# Autodesk Inventor assembly: CNC-FullAssembly
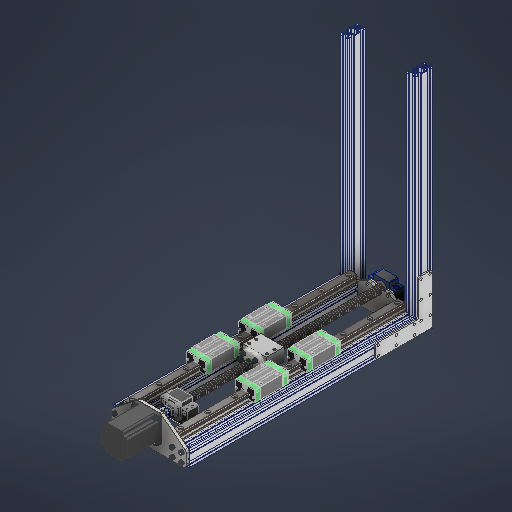
[picture p0: Inventor's stored thumbnail of the model, 512x512]
Saved by Autodesk Inventor 2026.2 (Build 302298000, 298)
## iProperties
Created: 2026-06-14
Part Number: CNC-FullAssembly
Document SubType Name: Assembly
Designer: Kenji
Mass: 7911.16 g
Surface Area: 12466.7 cm^2
Volume: 1822.96 cm^3
Density: 4.33972 g/cm^3
Author: Kenji
## Documents named in this file (20)
- C:\Users\Kenji\Documents\GitHub\DiyCNC-\CNC-FullAssembly.iam
- C:\Users\Kenji\Documents\GitHub\DiyCNC-\COTS-Parts\40x40x500mm-Extrusion.ipt
- C:\Users\Kenji\Documents\GitHub\DiyCNC-\COTS-Parts\SFU1605-BallScrewNut.iam
- C:\Users\Kenji\Documents\GitHub\DiyCNC-\COTS-Parts\DSG16H-BallScrewFixtureBlock.ipt
- C:\Users\Kenji\Documents\GitHub\DiyCNC-\COTS-Parts\SFU1605-BallScrew500mm.ipt
- C:\Users\Kenji\Documents\GitHub\DiyCNC-\COTS-Parts\BK12-BallScrewStabilizer.iam
- C:\Users\Kenji\Documents\GitHub\DiyCNC-\COTS-Parts\HGR20R-LinearRail500mm.ipt
- C:\Users\Kenji\Documents\GitHub\DiyCNC-\COTS-Parts\HGH20-LinearRailCarriage.iam
- C:\Users\Kenji\Documents\GitHub\DiyCNC-\COTS-Parts\91274A131_M5x20mm.ipt
- C:\Users\Kenji\Documents\GitHub\DiyCNC-\COTS-Parts\91290A231-M5x15mm.ipt
- C:\Users\Kenji\Documents\GitHub\DiyCNC-\COTS-Parts\Nema23-StepperMotor.ipt
- C:\Users\Kenji\Documents\GitHub\DiyCNC-\COTS-Parts\MH2025-6.35x10mmCoupler.iam
- C:\Users\Kenji\Documents\GitHub\DiyCNC-\COTS-Parts\BF12-BallScrewStabilizer2.ipt
- C:\Users\Kenji\Documents\GitHub\DiyCNC-\CNC-000-StructureGusset1.ipt
- C:\Users\Kenji\Documents\GitHub\DiyCNC-\COTS-Parts\20x40x500mm-Extrusion.ipt
- C:\Users\Kenji\Documents\GitHub\DiyCNC-\CNC-001-StructureGusset2.ipt
- C:\Users\Kenji\Documents\GitHub\DiyCNC-\CNC-002-ShimStructureGusset2.ipt
- C:\Users\Kenji\Documents\GitHub\DiyCNC-\COTS-Parts\90576A104-M5-NylockNut.ipt
- C:\Users\Kenji\Documents\GitHub\DiyCNC-\COTS-Parts\91292A195-M5x45mm.ipt
- C:\Users\Kenji\Documents\GitHub\DiyCNC-\CNC-003-StructureGusset3.ipt
## Components (70 placed, 19 different names)
1. 40x40x500mm-Extrusion:1 — Mate:1, Mate:2, Flush:1, Flush:2, Flush:3, Angle:1, Mate:6, Mate:12, Flush:5, Flush:6, Angle:3, Angle:4, Mate:46, Flush:20, Flush:21, Mate:48, Mate:49, Mate:50, Flush:35
2. 40x40x500mm-Extrusion:2 — Flush:2, Flush:3, Mate:7, Angle:2, Mate:11, Flush:9, Mate:39, Mate:40, Mate:41, Flush:22, Mate:47, Flush:23, Flush:38
3. SFU1605-BallScrewNut:1 [sub-assembly] — Mate:3, Mate:4, Mate:5, Mate:8, Mate:21, Mate:22, Mate:23, Mate:24, Mate:25, Mate:26, Mate:27
4. DSG16H-BallScrewFixtureBlock:1 — Mate:3, Mate:4, Mate:5, Angle:1, Mate:6, Mate:7, Flush:14, Mate:20
5. SFU1605-BallScrew500mm:1 — Mate:8, Mate:9, Mate:10, Mate:30, Mate:34, Mate:35, Mate:36
6. BK12-BallScrewStabilizer:1 [sub-assembly] — Mate:9, Mate:10, Angle:2
7. HGR20R-LinearRail500mm:1 — Mate:12, Flush:5, Flush:6, Flush:7, Flush:8, Mate:13, Mate:14, Mate:17, Mate:28, Mate:29, Mate:37
8. HGR20R-LinearRail500mm:2 — Mate:11, Flush:7, Flush:8, Flush:9, Mate:15, Mate:16, Mate:19
9. HGH20-LinearRailCarriage:1 [sub-assembly] — Mate:13, Mate:14, Flush:10, Flush:11, Mate:18, Flush:14
10. HGH20-LinearRailCarriage:2 [sub-assembly] — Mate:19, Flush:12, Flush:13
11. HGH20-LinearRailCarriage:3 [sub-assembly] — Mate:15, Mate:16, Flush:10, Flush:12, Mate:20
12. HGH20-LinearRailCarriage:4 [sub-assembly] — Mate:17, Flush:11, Mate:18, Flush:13
13. 91274A131_M5x20mm:1 — Mate:21, Mate:22, Flush:17, Flush:18
14. 91274A131_M5x20mm:2 — Mate:26, Flush:15, Flush:16
15. 91274A131_M5x20mm:3 — Mate:27, Flush:15
16. 91274A131_M5x20mm:4 — Mate:25, Flush:16, Flush:17
17. 91274A131_M5x20mm:5 — Mate:23, Flush:18, Flush:19
18. 91274A131_M5x20mm:6 — Mate:24, Flush:19
19. Nema23-StepperMotor:1 — Mate:32, Angle:3, Mate:33, Mate:59, Mate:60, Mate:61, Mate:62, Mate:63
20. MH2025-6.35x10mmCoupler:1 [sub-assembly] — Mate:30, Mate:32, Mate:33, Mate:34
21. BF12-BallScrewStabilizer2:1 — Mate:35, Mate:36, Angle:4, Mate:37, Mate:56, Mate:57, Mate:58
22. CNC-000-StructureGusset1:1 — Mate:39, Mate:40, Mate:41, Mate:42, Mate:43, Mate:44, Mate:45, Mate:65
23. 20x40x500mm-Extrusion:1 — Mate:46, Flush:20, Flush:21, Mate:71, Mate:72, Mate:73, Mate:74, Mate:75, Flush:36
24. 20x40x500mm-Extrusion:2 — Flush:22, Mate:47, Flush:23, Mate:69, Mate:70, Mate:76, Flush:37
25. CNC-001-StructureGusset2:1 — Mate:48, Mate:49, Mate:50, Mate:51, Mate:52, Mate:53, Mate:54, Mate:55
26. 91290A231-M5x15mm:27 — Mate:51, Mate:52, Flush:25, Flush:26
27. 91290A231-M5x15mm:28 — Mate:54, Flush:24, Flush:25
28. 91290A231-M5x15mm:29 — Mate:55, Flush:24
29. 91290A231-M5x15mm:30 — Mate:53, Flush:26
30. CNC-002-ShimStructureGusset2:1 — Mate:56, Mate:57, Mate:58
31. 91274A131_M5x20mm:7 — Mate:60, Flush:29, Mate:67
32. 91274A131_M5x20mm:8 — Mate:62, Mate:63, Flush:27, Mate:68
33. 91274A131_M5x20mm:9 — Mate:59, Flush:28, Flush:29, Mate:64
34. 91274A131_M5x20mm:10 — Mate:61, Flush:27, Flush:28, Mate:66
35. 90576A104-M5-NylockNut:1 — Mate:64, Mate:65, Flush:32
36. 90576A104-M5-NylockNut:2 — Mate:66, Flush:30
37. 90576A104-M5-NylockNut:3 — Mate:68, Flush:30, Flush:31
38. 90576A104-M5-NylockNut:4 — Mate:67, Flush:31, Flush:32
39. 91292A195-M5x45mm:1 — Mate:69, Flush:33, Flush:34
40. 91292A195-M5x45mm:2 — Mate:70, Flush:34
41. 91292A195-M5x45mm:3 — Mate:72, Mate:73
42. 91292A195-M5x45mm:4 — Mate:71, Mate:74, Flush:33
43. CNC-003-StructureGusset3:1 — Mate:75, Flush:35, Flush:36
44. CNC-003-StructureGusset3:2 — Mate:76, Flush:37, Flush:38
45. 91290A231-M5x15mm:1 — Mate:28, Mate:29
46. 91290A231-M5x15mm:2
47. 91290A231-M5x15mm:3
48. 91290A231-M5x15mm:4
49. 91290A231-M5x15mm:5
50. 91290A231-M5x15mm:6
51. 91290A231-M5x15mm:7
52. 91290A231-M5x15mm:8
53. 91290A231-M5x15mm:9
54. 91290A231-M5x15mm:10
55. 91290A231-M5x15mm:11
56. 91290A231-M5x15mm:12
57. 91290A231-M5x15mm:13
58. 91290A231-M5x15mm:14
59. 91290A231-M5x15mm:15
60. 91290A231-M5x15mm:16
61. 91290A231-M5x15mm:17
62. 91290A231-M5x15mm:18
63. 91290A231-M5x15mm:20 — Mate:44, Mate:45
64. 91290A231-M5x15mm:21
65. 91290A231-M5x15mm:22
66. 91290A231-M5x15mm:23
67. 91290A231-M5x15mm:19 — Mate:42, Mate:43
68. 91290A231-M5x15mm:24
69. 91290A231-M5x15mm:25
70. 91290A231-M5x15mm:26
## Component patterns: (18 elements, first: 91290A231-M5x15mm:1), (4 elements, first: 91290A231-M5x15mm:20), (4 elements, first: 91290A231-M5x15mm:19)
## Relationships (115: Mate 74, Flush 37, Angle 4)
- Mate:1 (-20 mm): 40x40x500mm-Extrusion:1
- Mate:2 (-20 mm): 40x40x500mm-Extrusion:1
- Flush:1 (-250 mm): 40x40x500mm-Extrusion:1
- Flush:2: 40x40x500mm-Extrusion:1 ↔ 40x40x500mm-Extrusion:2
- Flush:3: 40x40x500mm-Extrusion:1 ↔ 40x40x500mm-Extrusion:2
- Mate:3: SFU1605-BallScrewNut:1 ↔ DSG16H-BallScrewFixtureBlock:1
- Mate:4: SFU1605-BallScrewNut:1 ↔ DSG16H-BallScrewFixtureBlock:1
- Mate:5: SFU1605-BallScrewNut:1 ↔ DSG16H-BallScrewFixtureBlock:1
- Angle:1 (0 deg): 40x40x500mm-Extrusion:1 ↔ DSG16H-BallScrewFixtureBlock:1
- Mate:6 (18 mm): 40x40x500mm-Extrusion:1 ↔ DSG16H-BallScrewFixtureBlock:1
- Mate:7 (18 mm): 40x40x500mm-Extrusion:2 ↔ DSG16H-BallScrewFixtureBlock:1
- Mate:8: SFU1605-BallScrewNut:1 ↔ SFU1605-BallScrew500mm:1
- Mate:9: SFU1605-BallScrew500mm:1 ↔ BK12-BallScrewStabilizer:1
- Mate:10: SFU1605-BallScrew500mm:1 ↔ BK12-BallScrewStabilizer:1
- Angle:2 (0 deg): 40x40x500mm-Extrusion:2 ↔ BK12-BallScrewStabilizer:1
- Mate:11: 40x40x500mm-Extrusion:2 ↔ HGR20R-LinearRail500mm:2
- Mate:12: 40x40x500mm-Extrusion:1 ↔ HGR20R-LinearRail500mm:1
- Flush:5: 40x40x500mm-Extrusion:1 ↔ HGR20R-LinearRail500mm:1
- Flush:6: 40x40x500mm-Extrusion:1 ↔ HGR20R-LinearRail500mm:1
- Flush:7: HGR20R-LinearRail500mm:1 ↔ HGR20R-LinearRail500mm:2
- Flush:8: HGR20R-LinearRail500mm:1 ↔ HGR20R-LinearRail500mm:2
- Flush:9: 40x40x500mm-Extrusion:2 ↔ HGR20R-LinearRail500mm:2
- Mate:13: HGR20R-LinearRail500mm:1 ↔ HGH20-LinearRailCarriage:1
- Mate:14: HGR20R-LinearRail500mm:1 ↔ HGH20-LinearRailCarriage:1
- Mate:15: HGR20R-LinearRail500mm:2 ↔ HGH20-LinearRailCarriage:3
- Mate:16: HGR20R-LinearRail500mm:2 ↔ HGH20-LinearRailCarriage:3
- Flush:10: HGH20-LinearRailCarriage:1 ↔ HGH20-LinearRailCarriage:3
- Mate:17: HGR20R-LinearRail500mm:1 ↔ HGH20-LinearRailCarriage:4
- Flush:11: HGH20-LinearRailCarriage:1 ↔ HGH20-LinearRailCarriage:4
- Mate:18 (40 mm): HGH20-LinearRailCarriage:1 ↔ HGH20-LinearRailCarriage:4
- Mate:19: HGR20R-LinearRail500mm:2 ↔ HGH20-LinearRailCarriage:2
- Flush:12: HGH20-LinearRailCarriage:2 ↔ HGH20-LinearRailCarriage:3
- Flush:13: HGH20-LinearRailCarriage:2 ↔ HGH20-LinearRailCarriage:4
- Flush:14: DSG16H-BallScrewFixtureBlock:1 ↔ HGH20-LinearRailCarriage:1
- Mate:20: DSG16H-BallScrewFixtureBlock:1 ↔ HGH20-LinearRailCarriage:3
- Mate:21: SFU1605-BallScrewNut:1 ↔ 91274A131_M5x20mm:1
- Mate:22: SFU1605-BallScrewNut:1 ↔ 91274A131_M5x20mm:1
- Mate:23: SFU1605-BallScrewNut:1 ↔ 91274A131_M5x20mm:5
- Mate:24: SFU1605-BallScrewNut:1 ↔ 91274A131_M5x20mm:6
- Mate:25: SFU1605-BallScrewNut:1 ↔ 91274A131_M5x20mm:4
- Mate:26: SFU1605-BallScrewNut:1 ↔ 91274A131_M5x20mm:2
- Mate:27: SFU1605-BallScrewNut:1 ↔ 91274A131_M5x20mm:3
- Flush:15: 91274A131_M5x20mm:2 ↔ 91274A131_M5x20mm:3
- Flush:16: 91274A131_M5x20mm:2 ↔ 91274A131_M5x20mm:4
- Flush:17: 91274A131_M5x20mm:1 ↔ 91274A131_M5x20mm:4
- Flush:18: 91274A131_M5x20mm:1 ↔ 91274A131_M5x20mm:5
- Flush:19: 91274A131_M5x20mm:5 ↔ 91274A131_M5x20mm:6
- Mate:28: HGR20R-LinearRail500mm:1 ↔ 91290A231-M5x15mm:1
- Mate:29: HGR20R-LinearRail500mm:1 ↔ 91290A231-M5x15mm:1
- Mate:30: SFU1605-BallScrew500mm:1 ↔ MH2025-6.35x10mmCoupler:1
- Mate:32: Nema23-StepperMotor:1 ↔ MH2025-6.35x10mmCoupler:1
- Angle:3 (0 deg): 40x40x500mm-Extrusion:1 ↔ Nema23-StepperMotor:1
- Mate:33 (2 mm): Nema23-StepperMotor:1 ↔ MH2025-6.35x10mmCoupler:1
- Mate:34 (2 mm): SFU1605-BallScrew500mm:1 ↔ MH2025-6.35x10mmCoupler:1
- Mate:35: SFU1605-BallScrew500mm:1 ↔ BF12-BallScrewStabilizer2:1
- Mate:36: SFU1605-BallScrew500mm:1 ↔ BF12-BallScrewStabilizer2:1
- Angle:4 (0 deg): 40x40x500mm-Extrusion:1 ↔ BF12-BallScrewStabilizer2:1
- Mate:37 (9.525 mm): HGR20R-LinearRail500mm:1 ↔ BF12-BallScrewStabilizer2:1
- Mate:39: 40x40x500mm-Extrusion:2 ↔ CNC-000-StructureGusset1:1
- Mate:40: 40x40x500mm-Extrusion:2 ↔ CNC-000-StructureGusset1:1
- Mate:41: 40x40x500mm-Extrusion:2 ↔ CNC-000-StructureGusset1:1
- Mate:42: CNC-000-StructureGusset1:1 ↔ 91290A231-M5x15mm:19
- Mate:43: CNC-000-StructureGusset1:1 ↔ 91290A231-M5x15mm:19
- Mate:44: CNC-000-StructureGusset1:1 ↔ 91290A231-M5x15mm:20
- Mate:45: CNC-000-StructureGusset1:1 ↔ 91290A231-M5x15mm:20
- Mate:46: 40x40x500mm-Extrusion:1 ↔ 20x40x500mm-Extrusion:1
- Flush:20: 40x40x500mm-Extrusion:1 ↔ 20x40x500mm-Extrusion:1
- Flush:21: 40x40x500mm-Extrusion:1 ↔ 20x40x500mm-Extrusion:1
- Flush:22: 40x40x500mm-Extrusion:2 ↔ 20x40x500mm-Extrusion:2
- Mate:47: 40x40x500mm-Extrusion:2 ↔ 20x40x500mm-Extrusion:2
- Flush:23: 40x40x500mm-Extrusion:2 ↔ 20x40x500mm-Extrusion:2
- Mate:48: 40x40x500mm-Extrusion:1 ↔ CNC-001-StructureGusset2:1
- Mate:49: 40x40x500mm-Extrusion:1 ↔ CNC-001-StructureGusset2:1
- Mate:50: 40x40x500mm-Extrusion:1 ↔ CNC-001-StructureGusset2:1
- Mate:51: CNC-001-StructureGusset2:1 ↔ 91290A231-M5x15mm:27
- Mate:52: CNC-001-StructureGusset2:1 ↔ 91290A231-M5x15mm:27
- Mate:53: CNC-001-StructureGusset2:1 ↔ 91290A231-M5x15mm:30
- Mate:54: CNC-001-StructureGusset2:1 ↔ 91290A231-M5x15mm:28
- Mate:55: CNC-001-StructureGusset2:1 ↔ 91290A231-M5x15mm:29
- Flush:24: 91290A231-M5x15mm:28 ↔ 91290A231-M5x15mm:29
- Flush:25: 91290A231-M5x15mm:27 ↔ 91290A231-M5x15mm:28
- Flush:26: 91290A231-M5x15mm:27 ↔ 91290A231-M5x15mm:30
- Mate:56: BF12-BallScrewStabilizer2:1 ↔ CNC-002-ShimStructureGusset2:1
- Mate:57: BF12-BallScrewStabilizer2:1 ↔ CNC-002-ShimStructureGusset2:1
- Mate:58: BF12-BallScrewStabilizer2:1 ↔ CNC-002-ShimStructureGusset2:1
- Mate:59: Nema23-StepperMotor:1 ↔ 91274A131_M5x20mm:9
- Mate:60: Nema23-StepperMotor:1 ↔ 91274A131_M5x20mm:7
- Mate:61: Nema23-StepperMotor:1 ↔ 91274A131_M5x20mm:10
- Mate:62: Nema23-StepperMotor:1 ↔ 91274A131_M5x20mm:8
- Mate:63: Nema23-StepperMotor:1 ↔ 91274A131_M5x20mm:8
- Flush:27: 91274A131_M5x20mm:8 ↔ 91274A131_M5x20mm:10
- Flush:28: 91274A131_M5x20mm:9 ↔ 91274A131_M5x20mm:10
- Flush:29: 91274A131_M5x20mm:7 ↔ 91274A131_M5x20mm:9
- Mate:64: 91274A131_M5x20mm:9 ↔ 90576A104-M5-NylockNut:1
- Mate:65: CNC-000-StructureGusset1:1 ↔ 90576A104-M5-NylockNut:1
- Mate:66: 91274A131_M5x20mm:10 ↔ 90576A104-M5-NylockNut:2
- Mate:67: 91274A131_M5x20mm:7 ↔ 90576A104-M5-NylockNut:4
- Mate:68: 91274A131_M5x20mm:8 ↔ 90576A104-M5-NylockNut:3
- Flush:30: 90576A104-M5-NylockNut:2 ↔ 90576A104-M5-NylockNut:3
- Flush:31: 90576A104-M5-NylockNut:3 ↔ 90576A104-M5-NylockNut:4
- Flush:32: 90576A104-M5-NylockNut:1 ↔ 90576A104-M5-NylockNut:4
- Mate:69: 20x40x500mm-Extrusion:2 ↔ 91292A195-M5x45mm:1
- Mate:70: 20x40x500mm-Extrusion:2 ↔ 91292A195-M5x45mm:2
- Mate:71: 20x40x500mm-Extrusion:1 ↔ 91292A195-M5x45mm:4
- Mate:72: 20x40x500mm-Extrusion:1 ↔ 91292A195-M5x45mm:3
- Mate:73: 20x40x500mm-Extrusion:1 ↔ 91292A195-M5x45mm:3
- Mate:74: 20x40x500mm-Extrusion:1 ↔ 91292A195-M5x45mm:4
- Flush:33: 91292A195-M5x45mm:1 ↔ 91292A195-M5x45mm:4
- Flush:34: 91292A195-M5x45mm:1 ↔ 91292A195-M5x45mm:2
- Mate:75: 20x40x500mm-Extrusion:1 ↔ CNC-003-StructureGusset3:1
- Flush:35 (4.225 mm): 40x40x500mm-Extrusion:1 ↔ CNC-003-StructureGusset3:1
- Flush:36 (-4.225 mm): 20x40x500mm-Extrusion:1 ↔ CNC-003-StructureGusset3:1
- Mate:76: 20x40x500mm-Extrusion:2 ↔ CNC-003-StructureGusset3:2
- Flush:37 (-4.225 mm): 20x40x500mm-Extrusion:2 ↔ CNC-003-StructureGusset3:2
- Flush:38 (4.225 mm): 40x40x500mm-Extrusion:2 ↔ CNC-003-StructureGusset3:2
